# Autodesk Inventor assembly: MBD_Lmotorbar
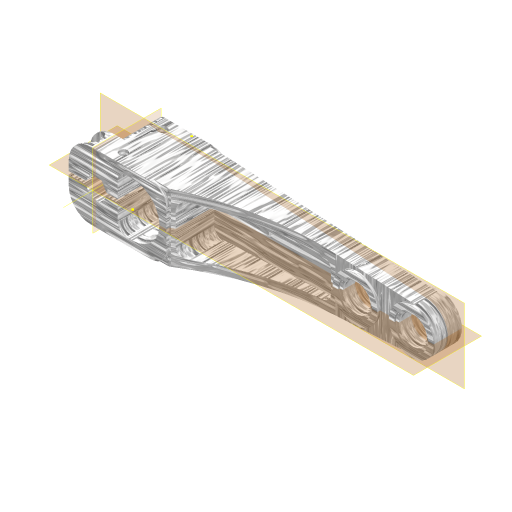
[picture p0: Inventor's stored thumbnail of the model, 512x512]
Saved by Autodesk Inventor 2023 (Build 270158000, 158)
## iProperties
Created: 2022-06-23
Part Number: MBD_Lmotorbar
Document SubType Name: Assembly
Designer: BioRoLaT470S
Mass: 52.4138 g
Surface Area: 120.675 cm^2
Volume: 18.6526 cm^3
Density: 2.81 g/cm^3
Author: BioRoLaT470S
## Documents named in this file (2)
- C:\Users\guanlunlu\Desktop\MBD_CORGI\CAD\MBD_Lmotorbar.iam
- C:\Users\guanlunlu\Desktop\MBD_CORGI\R100_properties\組合檔_v4\Rmotor_v2(open).ipt
## Components (1 placed, 1 different names)
1. Rmotor_v2(open):1 — Mate:1, Mate:2, Flush:1
## Relationships (3: Mate 2, Flush 1)
- Mate:1: Rmotor_v2(open):1
- Mate:2: Rmotor_v2(open):1
- Flush:1: Rmotor_v2(open):1
